# Autodesk Inventor assembly: cellSTORM_v5_ELECTRONICS
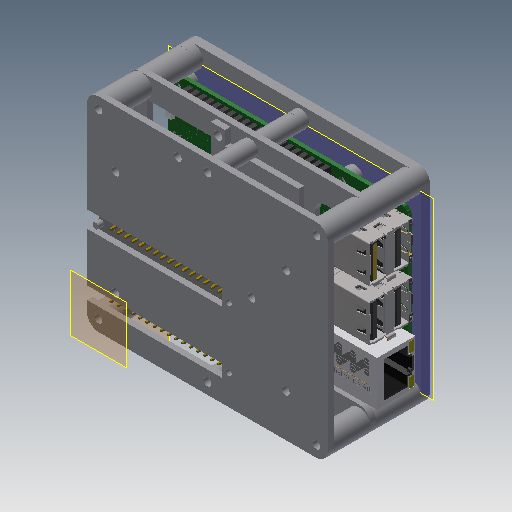
[picture p0: Inventor's stored thumbnail of the model, 512x512]
Saved by Autodesk Inventor 2019.4 (Build 234330000, 330)
## iProperties
Created: 2020-05-06
Part Number: cellSTORM_v5_ELECTRONICS
Document SubType Name: Assembly
Designer: diederichbenedict
Author: diederichbenedict
## Documents named in this file (7)
- C:\Users\diederichbenedict\Dropbox\Dokumente\Promotion\PROJECTS\STORMoChip\GITHUB\CAD\Nanoscopy-on-the-cheap\Workspace\cellSTORM_v5_ELECTRONICS.iam
- C:\Users\diederichbenedict\Dropbox\Dokumente\Promotion\PROJECTS\STORMoChip\GITHUB\CAD\Nanoscopy-on-the-cheap\Workspace\cellSTORM_v5_Electronicbox_upperlayer.ipt
- C:\Users\diederichbenedict\Dropbox\Dokumente\Promotion\PROJECTS\STORMoChip\GITHUB\CAD\Nanoscopy-on-the-cheap\Workspace\cellSTORM_v5_Electronicbox_midlayer.ipt
- C:\Users\diederichbenedict\Dropbox\Dokumente\Promotion\PROJECTS\STORMoChip\GITHUB\CAD\Nanoscopy-on-the-cheap\Workspace\cellSTORM_v5_Electronicbox.ipt
- C:\Users\diederichbenedict\Dropbox\Dokumente\Promotion\PROJECTS\STORMoChip\GITHUB\CAD\Nanoscopy-on-the-cheap\Workspace\00_cellstorm_Amplifier.ipt
- C:\Users\diederichbenedict\Dropbox\Dokumente\Promotion\PROJECTS\STORMoChip\GITHUB\CAD\Nanoscopy-on-the-cheap\Workspace\ESP\00_ESP32.iam
- C:\Users\diederichbenedict\Dropbox\Dokumente\Promotion\PROJECTS\STORMoChip\GITHUB\CAD\Nanoscopy-on-the-cheap\Workspace\Raspi\00_Raspi.ipt
## Components (6 placed, 6 different names)
1. cellSTORM_v5_Electronicbox_upperlayer:1
2. cellSTORM_v5_Electronicbox_midlayer:1
3. cellSTORM_v5_Electronicbox:1
4. 00_cellstorm_Amplifier:1
5. 00_ESP32:1 [sub-assembly]
6. 00_Raspi:1
## Relationships (9: Flush 5, Mate 2, Insert 1, Angle 1)
- [Insert]: cellSTORM_v5_Electronicbox_upperlayer:1 ↔ cellSTORM_v5_Electronicbox_midlayer:1
- [Flush]: cellSTORM_v5_Electronicbox_midlayer:1 ↔ cellSTORM_v5_Electronicbox:1
- [Mate]: cellSTORM_v5_Electronicbox_midlayer:1 ↔ 00_cellstorm_Amplifier:1
- [Flush] (-1 mm): cellSTORM_v5_Electronicbox_midlayer:1 ↔ 00_cellstorm_Amplifier:1
- [Flush]: cellSTORM_v5_Electronicbox:1 ↔ 00_Raspi:1
- [Flush] (3.25 mm): cellSTORM_v5_Electronicbox:1 ↔ 00_Raspi:1
- [Mate] (1 mm): cellSTORM_v5_Electronicbox_midlayer:1 ↔ 00_ESP32:1
- [Angle] (0 deg): cellSTORM_v5_Electronicbox_midlayer:1 ↔ 00_ESP32:1
- [Flush] (-5 mm): cellSTORM_v5_Electronicbox_midlayer:1 ↔ 00_ESP32:1
